# Autodesk Inventor assembly: FullAssembly
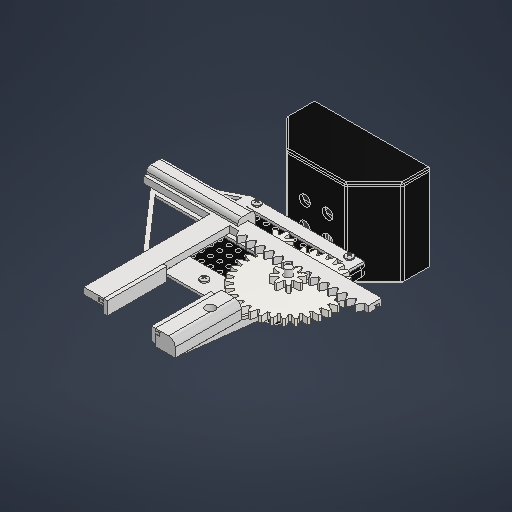
[picture p0: Inventor's stored thumbnail of the model, 512x512]
Saved by Autodesk Inventor 2026.1 (Build 301233000, 233)
## iProperties
Created: 2025-10-14
Part Number: FullAssembly
Document SubType Name: Assembly
Designer: alexj
Mass: 366.358 g
Surface Area: 1579.05 cm^2
Volume: 245.213 cm^3
Density: 1.49404 g/cm^3
Author: alexj
## Documents named in this file (11)
- C:\Users\rhema\ENG course\P1\Models\Final\FullAssembly.iam
- C:\Users\rhema\ENG course\P1\Models\Final\End Effector Platform.iam
- C:\Users\rhema\ENG course\P1\Models\Final\Steel M3x16 Pan Head Screw.ipt
- C:\Users\rhema\ENG course\P1\Models\Final\BasePlate.ipt
- C:\Users\rhema\ENG course\P1\Models\Final\CenterGear.ipt
- C:\Users\rhema\ENG course\P1\Models\Final\LargeStackedGear.ipt
- C:\Users\rhema\ENG course\P1\Models\Final\PinionGear.ipt
- C:\Users\rhema\ENG course\P1\Models\Final\Rack 6.5mm 10mm short.ipt
- C:\Users\rhema\ENG course\P1\Models\Final\Base Gripper Support.ipt
- C:\Users\rhema\ENG course\P1\Models\Final\Rack Gripper.ipt
- C:\Users\rhema\ENG course\P1\Fasteners\Steel M3 Hex Nut.ipt
## Components (19 placed, 8 different names)
1. End Effector Platform:2 [sub-assembly] — Mate:1, Mate:2, Mate:8, Angle:1, Mate:17, Insert:5, Insert:6, Insert:7
2. Steel M3x16 Pan Head Screw:2 — Mate:4, Mate:20, Angle:2
3. Steel M3x16 Pan Head Screw:4 — Mate:7, Mate:18, Angle:3
4. BasePlate:1 — Mate:1, Mate:2, Mate:4, Mate:7, Mate:9, Mate:10, Mate:11, Mate:12, Mate:16, Mate:17, Mate:18, Mate:19, Mate:20, Flush:1, Mate:24, Flush:7, Flush:8, Flush:11, Insert:1, Insert:2
5. Spur Gear1:1 — Mate:8, Mate:9, Angle:1, Rotation:1
6. Spur Gear1:2 — Mate:10, Mate:11, Rotation:1, Mate:13, Rotation:2
7. Spur Gear1:3 — Mate:12, Mate:13, Rotation:2, Rotation/Translation:1
8. Rack 6.5mm 10mm short:1 — Rotation/Translation:1, Flush:1, Flush:9
9. Steel M3x16 Pan Head Screw:5 — Mate:16, Mate:19, Angle:4
10. Base Gripper Support:1 — Flush:11, Insert:3, Insert:4
11. Rack Gripper:1 — Flush:9, Flush:10
12. Rack Gripper:3 — Mate:24, Flush:7, Flush:8, Flush:10
13. Steel M3x16 Pan Head Screw:6 — Angle:5, Insert:1
14. Steel M3x16 Pan Head Screw:7 — Angle:6, Insert:2
15. Steel M3 Hex Nut:1 — Insert:4, Angle:7
16. Steel M3 Hex Nut:3 — Insert:3, Angle:8
17. Steel M3 Hex Nut:4 — Insert:6, Angle:9
18. Steel M3 Hex Nut:5 — Insert:5, Angle:10
19. Steel M3 Hex Nut:6 — Insert:7, Angle:11
## Relationships (43: Mate 16, Angle 11, Insert 7, Flush 6, RelateRotation 2, RelateRotateTranslate 1)
- Mate:1: End Effector Platform:2 ↔ BasePlate:1
- Mate:2: End Effector Platform:2 ↔ BasePlate:1
- Mate:4: Steel M3x16 Pan Head Screw:2 ↔ BasePlate:1
- Mate:7: Steel M3x16 Pan Head Screw:4 ↔ BasePlate:1
- Mate:8: End Effector Platform:2 ↔ Spur Gear1:1
- Mate:9: BasePlate:1 ↔ Spur Gear1:1
- Angle:1 (720 deg): End Effector Platform:2 ↔ Spur Gear1:1
- Mate:10: BasePlate:1 ↔ Spur Gear1:2
- Mate:11: BasePlate:1 ↔ Spur Gear1:2
- Rotation:1 [RelateRotation] (0.25 ul): Spur Gear1:1 ↔ Spur Gear1:2
- Mate:12: BasePlate:1 ↔ Spur Gear1:3
- Mate:13: Spur Gear1:2 ↔ Spur Gear1:3
- Rotation:2 [RelateRotation] (1 ul): Spur Gear1:2 ↔ Spur Gear1:3
- Rotation/Translation:1 [RelateRotateTranslate] (55.072 mm): Spur Gear1:3 ↔ Rack 6.5mm 10mm short:1
- Mate:16: BasePlate:1 ↔ Steel M3x16 Pan Head Screw:5
- Mate:17: End Effector Platform:2 ↔ BasePlate:1
- Mate:18: Steel M3x16 Pan Head Screw:4 ↔ BasePlate:1
- Mate:19: BasePlate:1 ↔ Steel M3x16 Pan Head Screw:5
- Mate:20: Steel M3x16 Pan Head Screw:2 ↔ BasePlate:1
- Flush:1: BasePlate:1 ↔ Rack 6.5mm 10mm short:1
- Mate:24: BasePlate:1 ↔ Rack Gripper:3
- Flush:7: BasePlate:1 ↔ Rack Gripper:3
- Flush:8: BasePlate:1 ↔ Rack Gripper:3
- Flush:9: Rack 6.5mm 10mm short:1 ↔ Rack Gripper:1
- Flush:10: Rack Gripper:1 ↔ Rack Gripper:3
- Angle:2 (0 deg): Steel M3x16 Pan Head Screw:2
- Angle:3 (0 deg): Steel M3x16 Pan Head Screw:4
- Angle:4 (0 deg): Steel M3x16 Pan Head Screw:5
- Flush:11: BasePlate:1 ↔ Base Gripper Support:1
- Angle:5 (0 deg): Steel M3x16 Pan Head Screw:6
- Angle:6 (0 deg): Steel M3x16 Pan Head Screw:7
- Insert:1: BasePlate:1 ↔ Steel M3x16 Pan Head Screw:6
- Insert:2: BasePlate:1 ↔ Steel M3x16 Pan Head Screw:7
- Insert:3: Base Gripper Support:1 ↔ Steel M3 Hex Nut:3
- Insert:4: Base Gripper Support:1 ↔ Steel M3 Hex Nut:1
- Insert:5: End Effector Platform:2 ↔ Steel M3 Hex Nut:5
- Insert:6: End Effector Platform:2 ↔ Steel M3 Hex Nut:4
- Insert:7: End Effector Platform:2 ↔ Steel M3 Hex Nut:6
- Angle:7 (0 deg): Steel M3 Hex Nut:1
- Angle:8 (0 deg): Steel M3 Hex Nut:3
- Angle:9 (0 deg): Steel M3 Hex Nut:4
- Angle:10 (0 deg): Steel M3 Hex Nut:5
- Angle:11 (0 deg): Steel M3 Hex Nut:6
